# Autodesk Inventor assembly: Assembly1
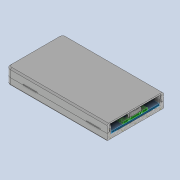
[picture p0: Inventor's stored thumbnail of the model, 180x180]
Saved by Autodesk Inventor 2022 (Build 260153000, 153)
## iProperties
Created: 2025-09-23
Part Number: Assembly1
Document SubType Name: Assembly
Designer: 1234
Author: 1234
## Documents named in this file (4)
- C:\Users\1234\Dropbox\Giorgio_Mac\PPS (pascon piccone sacchiero)\componenti\hub\Assembly1.iam
- C:\Users\1234\Dropbox\Giorgio_Mac\PPS (pascon piccone sacchiero)\PCB\PCB_hub_rev_0\PCB_hub_rev_0.iam
- C:\Users\1234\Dropbox\Giorgio_Mac\PPS (pascon piccone sacchiero)\componenti\hub\scatola_v2_sopra.ipt
- C:\Users\1234\Dropbox\Giorgio_Mac\PPS (pascon piccone sacchiero)\componenti\hub\scatola_v2_sotto.ipt
## Components (3 placed, 3 different names)
1. PCB_hub_rev_0:1 [sub-assembly] — Mate:1, Mate:3, Mate:4
2. scatola_v2_sopra:1 — Mate:2, Flush:1, Flush:2
3. scatola_v2_sotto:1 — Mate:1, Mate:2, Flush:1, Mate:3, Mate:4, Flush:2
## Relationships (6: Mate 4, Flush 2)
- Mate:1: PCB_hub_rev_0:1 ↔ scatola_v2_sotto:1
- Mate:2: scatola_v2_sopra:1 ↔ scatola_v2_sotto:1
- Flush:1: scatola_v2_sopra:1 ↔ scatola_v2_sotto:1
- Mate:3: PCB_hub_rev_0:1 ↔ scatola_v2_sotto:1
- Mate:4: PCB_hub_rev_0:1 ↔ scatola_v2_sotto:1
- Flush:2: scatola_v2_sopra:1 ↔ scatola_v2_sotto:1
